# Autodesk Inventor assembly: Сборка ручка упрощённая
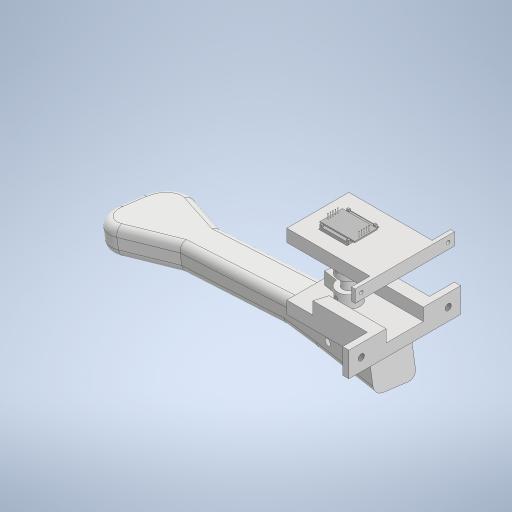
[picture p0: Inventor's stored thumbnail of the model, 512x512]
Saved by Autodesk Inventor 2023 (Build 270158000, 158)
## iProperties
Created: 2022-05-02
Part Number: Сборка ручка упрощённая
Document SubType Name: Assembly
Designer: User
Author: User
## Documents named in this file (10)
- D:\Стойка\VR-simulator-3D-models\Механизм ручки\Сборка ручка упрощённая.iam
- D:\Стойка\VR-simulator-3D-models\Механизм ручки\EAW.ipt
- D:\Стойка\VR-simulator-3D-models\Механизм ручки\Вал ручки.ipt
- D:\Стойка\VR-simulator-3D-models\Механизм ручки\Втулка энкодер.ipt
- D:\Стойка\VR-simulator-3D-models\Механизм ручки\Ручка.ipt
- D:\Стойка\VR-simulator-3D-models\Механизм ручки\Стенка.ipt
- D:\Стойка\VR-simulator-3D-models\Механизм ручки\Стопор.ipt
- D:\Стойка\VR-simulator-3D-models\Механизм ручки\Стенка энкодер.ipt
- D:\Стойка\VR-simulator-3D-models\Механизм ручки\М3х8.ipt
- D:\Стойка\VR-simulator-3D-models\Механизм ручки\Диск конец вала.ipt
## Components (9 placed, 9 different names)
1. EAW:1 — Цилиндрический:4, Совмещение:6, Совмещение:7
2. Вал ручки:1 — Цилиндрический:1, Совмещение:1, Цилиндрический:2, Цилиндрический:5, Совмещение:2, Цилиндрический:12, Совмещение:4, Совмещение:5
3. Втулка энкодер:1 — Цилиндрический:4, Совмещение:4, Совмещение:5, Совмещение:7
4. Ручка:1 — Цилиндрический:1, Совмещение:1
5. Стенка:1 — Заподлицо:1, Заподлицо:2, Цилиндрический:5, Совмещение:3
6. Стопор:1 — Цилиндрический:2, Совмещение:2, Совмещение:3
7. Стенка энкодер:1 — Заподлицо:1, Заподлицо:2, Совмещение:6
8. М3х8:1 — Цилиндрический:11, Цилиндрический:12
9. Диск конец вала:1 — Цилиндрический:11
## Relationships (15: Mate 7, CylindricalJoint 6, Flush 2)
- Цилиндрический:1 [CylindricalJoint]: Вал ручки:1 ↔ Ручка:1
- Совмещение:1 [Mate]: Вал ручки:1 ↔ Ручка:1
- Цилиндрический:2 [CylindricalJoint]: Вал ручки:1 ↔ Стопор:1
- Заподлицо:1 [Flush]: Стенка:1 ↔ Стенка энкодер:1
- Цилиндрический:4 [CylindricalJoint]: EAW:1 ↔ Втулка энкодер:1
- Заподлицо:2 [Flush]: Стенка:1 ↔ Стенка энкодер:1
- Цилиндрический:5 [CylindricalJoint]: Вал ручки:1 ↔ Стенка:1
- Совмещение:2 [Mate]: Вал ручки:1 ↔ Стопор:1
- Совмещение:3 [Mate]: Стенка:1 ↔ Стопор:1
- Цилиндрический:11 [CylindricalJoint]: М3х8:1 ↔ Диск конец вала:1
- Цилиндрический:12 [CylindricalJoint]: Вал ручки:1 ↔ М3х8:1
- Совмещение:4 [Mate]: Вал ручки:1 ↔ Втулка энкодер:1
- Совмещение:5 [Mate]: Вал ручки:1 ↔ Втулка энкодер:1
- Совмещение:6 [Mate]: EAW:1 ↔ Стенка энкодер:1
- Совмещение:7 [Mate]: EAW:1 ↔ Втулка энкодер:1
